# Autodesk Inventor assembly: MG-Verbindungsstrebe Links
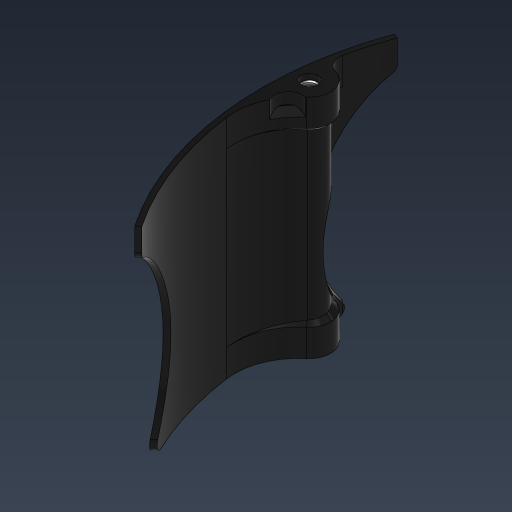
[picture p0: Inventor's stored thumbnail of the model, 512x512]
Saved by Autodesk Inventor 2023.1 (Build 271208000, 208)
## iProperties
Part Number: MG-Verbindungsstrebe Links
Material: Generisch
Document SubType Name: Assembly
Designer: rYan
Author: rYan
## Documents named in this file (3)
- D:\TIGERsGIT\mechanics-releases\v2024\Inventor\Robot\Electronics\MG-Verbindungsstrebe Links.iam
- D:\TIGERsGIT\mechanics-releases\v2024\Inventor\Robot\Electronics\Verbindungsstrebe Links.ipt
- D:\TIGERsGIT\mechanics-releases\v2024\Inventor\Inhaltscenter\de-DE\DIN 934\DIN 934 - M4 x 0,7.ipt
## Components (3 placed, 2 different names)
1. Verbindungsstrebe Links:1 — Fluchtend:1, Fluchtend:2, Fluchtend:3, Einfügen:1, Einfügen:2
2. DIN 934 - ersetzt durch DIN EN 24032/28673/28674 M4:1 — Einfügen:2
3. DIN 934 - ersetzt durch DIN EN 24032/28673/28674 M4:2 — Einfügen:1
## Relationships (5: Flush 3, Insert 2)
- Fluchtend:1 [Flush]: Verbindungsstrebe Links:1
- Fluchtend:2 [Flush]: Verbindungsstrebe Links:1
- Fluchtend:3 [Flush]: Verbindungsstrebe Links:1
- Einfügen:1 [Insert]: Verbindungsstrebe Links:1 ↔ DIN 934 - ersetzt durch DIN EN 24032/28673/28674 M4:2
- Einfügen:2 [Insert]: Verbindungsstrebe Links:1 ↔ DIN 934 - ersetzt durch DIN EN 24032/28673/28674 M4:1
